# Autodesk Inventor assembly: EnsamblajeVarillas
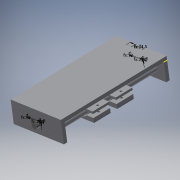
[picture p0: Inventor's stored thumbnail of the model, 180x180]
Saved by Autodesk Inventor 2017 (Build 210142000, 142)
## iProperties
Part Number: EnsamblajeVarillas
Material: Genérico
Document SubType Name: Assembly
Designer: osvaldo
Author: osvaldo
## Documents named in this file (7)
- C:\Users\osvaldo\Documents\Inventor\Eje Z\EnsamblajeVarillas.iam
- C:\Users\osvaldo\Documents\Inventor\Eje Z\Placa2.ipt
- C:\Users\osvaldo\Documents\Inventor\Eje Z\Varilla.ipt
- C:\Users\osvaldo\Documents\Inventor\Content Center Files\R2017\es-ES\DIN 976-1 A\DIN 976-1 - M8 x 160 - A.ipt
- C:\Users\osvaldo\Documents\Inventor\Eje Z\PiezaPeluda.ipt
- C:\Users\osvaldo\Documents\Inventor\Eje Z\Rodamiento.ipt
- C:\Users\osvaldo\Documents\Inventor\Eje Z\Placa.ipt
## Components (12 placed, 6 different names)
1. DIN 976-1 A M8 x 160:1 — De rotación:1
2. Placa2:1 — De rotación:1, Ángulo:3, Ángulo:4, Coincidencia:6, Coincidencia:7, Ángulo:5, Coincidencia:9, Coincidencia:10, Coincidencia:11, Coincidencia:12, Coincidencia:13
3. Placa2:2 — Coincidencia:8, Ángulo:6, Ángulo:7
4. Varilla:1 — Coincidencia:2, Coincidencia:4, Coincidencia:6, Coincidencia:8
5. Varilla:2 — Coincidencia:3, Coincidencia:5, Coincidencia:7, Coincidencia:14
6. PiezaPeluda:1 — Rígido:7, Rígido:6, Coincidencia:1, Coincidencia:4, Ángulo:4, Coincidencia:14
7. PiezaPeluda:2 — Rígido:4, Rígido:5, Coincidencia:1, Ángulo:3, Coincidencia:2, Coincidencia:3, Coincidencia:5
8. Rodamiento:1 — Rígido:4
9. Rodamiento:2 — Rígido:5
10. Rodamiento:3 — Rígido:7
11. Rodamiento:4 — Rígido:6
12. Placa:1 — Ángulo:5, Coincidencia:9, Coincidencia:10, Coincidencia:11, Coincidencia:12, Coincidencia:13, Ángulo:6, Ángulo:7
## Relationships (24: Mate 14, Angle 5, WeldJoint 4, RevoluteJoint 1)
- De rotación:1 [RevoluteJoint] (-5 mm): DIN 976-1 A M8 x 160:1 ↔ Placa2:1
- Rígido:4 [WeldJoint] (5 mm): PiezaPeluda:2 ↔ Rodamiento:1
- Rígido:5 [WeldJoint] (5 mm): PiezaPeluda:2 ↔ Rodamiento:2
- Rígido:7 [WeldJoint] (5 mm): PiezaPeluda:1 ↔ Rodamiento:3
- Rígido:6 [WeldJoint] (5 mm): PiezaPeluda:1 ↔ Rodamiento:4
- Coincidencia:1 [Mate] (10 mm): PiezaPeluda:1 ↔ PiezaPeluda:2
- Ángulo:3 [Angle] (0 deg): Placa2:1 ↔ PiezaPeluda:2
- Coincidencia:2 [Mate]: Varilla:1 ↔ PiezaPeluda:2
- Coincidencia:3 [Mate]: Varilla:2 ↔ PiezaPeluda:2
- Coincidencia:4 [Mate]: Varilla:1 ↔ PiezaPeluda:1
- Coincidencia:5 [Mate]: Varilla:2 ↔ PiezaPeluda:2
- Ángulo:4 [Angle] (0 deg): Placa2:1 ↔ PiezaPeluda:1
- Coincidencia:6 [Mate]: Placa2:1 ↔ Varilla:1
- Coincidencia:7 [Mate]: Placa2:1 ↔ Varilla:2
- Coincidencia:8 [Mate]: Placa2:2 ↔ Varilla:1
- Ángulo:5 [Angle] (0 deg): Placa2:1 ↔ Placa:1
- Coincidencia:9 [Mate]: Placa2:1 ↔ Placa:1
- Coincidencia:10 [Mate]: Placa2:1 ↔ Placa:1
- Coincidencia:11 [Mate]: Placa2:1 ↔ Placa:1
- Coincidencia:12 [Mate]: Placa2:1 ↔ Placa:1
- Coincidencia:13 [Mate]: Placa2:1 ↔ Placa:1
- Ángulo:6 [Angle] (0 deg): Placa2:2 ↔ Placa:1
- Ángulo:7 [Angle] (0 deg): Placa2:2 ↔ Placa:1
- Coincidencia:14 [Mate]: Varilla:2 ↔ PiezaPeluda:1
## Named parameters: scale = 1 mm
